# Autodesk Inventor assembly: DoubleSlipHR
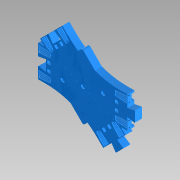
[picture p0: Inventor's stored thumbnail of the model, 180x180]
Saved by Autodesk Inventor 2021 (Build 250183000, 183)
## iProperties
Created: 2021-05-05
Part Number: DoubleSlipHR
Document SubType Name: Assembly
Designer: kumagai
Author: kumagai
## Documents named in this file (5)
- X:\Develop\CAD\PlaRails\DoubleSlip\DoubleSlipHR.iam
- X:\Develop\CAD\PlaRails\DoubleSlip\DoubleSlipHR.ipt
- X:\Develop\CAD\PlaRails\DoubleSlip\RailJointShortFemale.ipt
- X:\Develop\CAD\PlaRails\DoubleSlip\RailJointShortMale.ipt
- X:\Develop\CAD\PlaRails\DoubleSlip\DoubleSlipHR\DoubleSlipHR-45_H_H.ipt
## Components (6 placed, 3 different names)
1. DoubleSlipHR-45_H_H:3 — フラッシュ:1, フラッシュ:2, メイト:1, フラッシュ:3, フラッシュ:5, フラッシュ:7, フラッシュ:8, メイト:4, フラッシュ:9, メイト:5, メイト:6
2. DoubleSlipHR-45_H_H:4 — フラッシュ:9, メイト:5, メイト:6, フラッシュ:10, メイト:7, フラッシュ:11, メイト:8
3. RailJointShortFemale:1 — フラッシュ:7, フラッシュ:8, メイト:4
4. RailJointShortFemale:2 — フラッシュ:5, フラッシュ:10, メイト:7
5. RailJointShortMale:1 — フラッシュ:3, フラッシュ:11, メイト:8
6. RailJointShortMale:2 — フラッシュ:1, フラッシュ:2, メイト:1
## Relationships (15: Flush 9, Mate 6)
- フラッシュ:1 [Flush]: DoubleSlipHR-45_H_H:3 ↔ RailJointShortMale:2
- フラッシュ:2 [Flush]: DoubleSlipHR-45_H_H:3 ↔ RailJointShortMale:2
- メイト:1 [Mate]: DoubleSlipHR-45_H_H:3 ↔ RailJointShortMale:2
- フラッシュ:3 [Flush]: DoubleSlipHR-45_H_H:3 ↔ RailJointShortMale:1
- フラッシュ:5 [Flush]: DoubleSlipHR-45_H_H:3 ↔ RailJointShortFemale:2
- フラッシュ:7 [Flush]: DoubleSlipHR-45_H_H:3 ↔ RailJointShortFemale:1
- フラッシュ:8 [Flush]: DoubleSlipHR-45_H_H:3 ↔ RailJointShortFemale:1
- メイト:4 [Mate]: DoubleSlipHR-45_H_H:3 ↔ RailJointShortFemale:1
- フラッシュ:9 [Flush]: DoubleSlipHR-45_H_H:3 ↔ DoubleSlipHR-45_H_H:4
- メイト:5 [Mate]: DoubleSlipHR-45_H_H:3 ↔ DoubleSlipHR-45_H_H:4
- メイト:6 [Mate]: DoubleSlipHR-45_H_H:3 ↔ DoubleSlipHR-45_H_H:4
- フラッシュ:10 [Flush]: DoubleSlipHR-45_H_H:4 ↔ RailJointShortFemale:2
- メイト:7 [Mate]: DoubleSlipHR-45_H_H:4 ↔ RailJointShortFemale:2
- フラッシュ:11 [Flush]: DoubleSlipHR-45_H_H:4 ↔ RailJointShortMale:1
- メイト:8 [Mate]: DoubleSlipHR-45_H_H:4 ↔ RailJointShortMale:1
